# Autodesk Inventor assembly: ASSY,ROBOT,2026
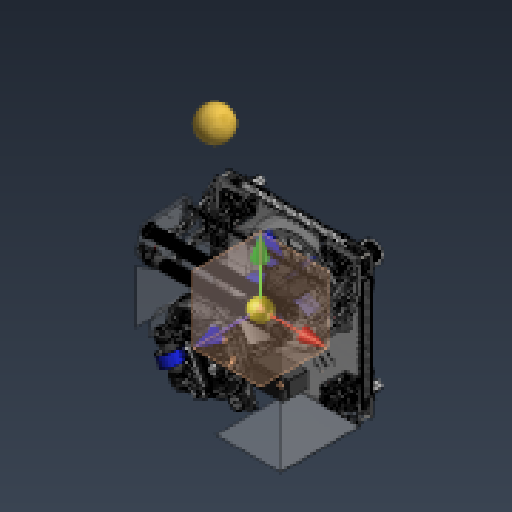
[picture p0: Inventor's stored thumbnail of the model, 512x512]
Saved by Autodesk Inventor 2026 (Build 300175050, 175E)
## iProperties
Created: 2026-01-24
Part Number: ASSY,ROBOT,2026
Document SubType Name: Assembly
Designer: Jthib
Mass: 50454.4 g
Surface Area: 114808 cm^2
Volume: 25614.5 cm^3
Density: 1.96976 g/cm^3
Author: Jthib
## Documents named in this file (11)
- C:\Users\Jthib\Documents\GitHub\2026-Robot-Mechanical\ASSY,ROBOT,2026.iam
- C:\Users\Jthib\Documents\GitHub\2026-Robot-Mechanical\Chassis\CHASSIS.iam
- C:\Users\Jthib\Documents\GitHub\2026-Robot-Mechanical\Spindexer\#Spindexer.iam
- C:\Users\Jthib\Documents\GitHub\2026-Robot-Mechanical\Shooter\Shooter - Front Motors\#SHOOTER.FRONT_MOTORS.iam
- C:\Users\Jthib\Documents\GitHub\2026-Robot-Mechanical\Shooter\Turret\#Turret.iam
- C:\Users\Jthib\Documents\GitHub\2026-Robot-Mechanical\Intake\ASSY,INTAKE.iam
- C:\Users\Jthib\Documents\GitHub\2026-Robot-Mechanical\#2_2026 Field CAD\GE-26900_ Fuel.ipt
- C:\Users\Jthib\Documents\GitHub\2026-Robot-Mechanical\Intake\PLATE,HOPPER,BACK.ipt
- C:\Users\Jthib\Documents\GitHub\2026-Robot-Mechanical\Intake\PLATE,HOPPER,FRONT.ipt
- C:\Users\Jthib\Documents\GitHub\2026-Robot-Mechanical\Intake\PLATE,HOPPER,BACK2.ipt
- C:\Users\Jthib\Documents\GitHub\2026-Robot-Mechanical\#1_CAD Library\Motors\MOTOR,REV,NEO,V1-1.ipt
## Components (11 placed, 10 different names)
1. CHASSIS:1 [sub-assembly] — Flush:1, Flush:2, Flush:3, Mate:9, Mate:10, Mate:11, Tangent:1, Mate:13, Mate:18, Mate:19, Mate:20, Mate:21, Flush:23, Mate:22, Flush:24, Mate:23, Mate:25, Flush:25
2. #Spindexer:1 [sub-assembly] — Mate:11, Mate:12, Tangent:1, Mate:13, Mate:15, Mate:16, Mate:17, Mate:18
3. #SHOOTER.FRONT_MOTORS:1 [sub-assembly] — Mate:9, Mate:10, Mate:12, Insert:1, Mate:14
4. #Turret:1 [sub-assembly] — Insert:1, Mate:14, Mate:15, Mate:16, Mate:17
5. ASSY,INTAKE:1 [sub-assembly] — Mate:19, Mate:20, Mate:21, Insert:2, Insert:3
6. GE-26900_ Fuel:1
7. PLATE,HOPPER,BACK:1 — Flush:23, Mate:22, Flush:24, Mate:24
8. PLATE,HOPPER,FRONT:1 — Mate:23, Mate:24
9. PLATE,HOPPER,BACK2:1 — Mate:25, Flush:25
10. MOTOR,REV,NEO,V1-1:1 — Insert:2
11. MOTOR,REV,NEO,V1-1:2 — Insert:3
## Relationships (27: Mate 17, Flush 6, Insert 3, Tangent 1)
- Flush:1 (-349.25 mm): CHASSIS:1
- Flush:2 (349.25 mm): CHASSIS:1
- Flush:3: CHASSIS:1
- Mate:9 (-190.5 mm): CHASSIS:1 ↔ #SHOOTER.FRONT_MOTORS:1
- Mate:10 (-190.5 mm): CHASSIS:1 ↔ #SHOOTER.FRONT_MOTORS:1
- Mate:11: CHASSIS:1 ↔ #Spindexer:1
- Mate:12 (79.375 mm): #Spindexer:1 ↔ #SHOOTER.FRONT_MOTORS:1
- Tangent:1: CHASSIS:1 ↔ #Spindexer:1
- Mate:13 (-304.8 mm): CHASSIS:1 ↔ #Spindexer:1
- Insert:1: #SHOOTER.FRONT_MOTORS:1 ↔ #Turret:1
- Mate:14: #SHOOTER.FRONT_MOTORS:1 ↔ #Turret:1
- Mate:15: #Spindexer:1 ↔ #Turret:1
- Mate:16: #Spindexer:1 ↔ #Turret:1
- Mate:17: #Spindexer:1 ↔ #Turret:1
- Mate:18: CHASSIS:1 ↔ #Spindexer:1
- Mate:19: CHASSIS:1 ↔ ASSY,INTAKE:1
- Mate:20: CHASSIS:1 ↔ ASSY,INTAKE:1
- Mate:21: CHASSIS:1 ↔ ASSY,INTAKE:1
- Flush:23: CHASSIS:1 ↔ PLATE,HOPPER,BACK:1
- Mate:22: CHASSIS:1 ↔ PLATE,HOPPER,BACK:1
- Flush:24: CHASSIS:1 ↔ PLATE,HOPPER,BACK:1
- Mate:23: CHASSIS:1 ↔ PLATE,HOPPER,FRONT:1
- Mate:24: PLATE,HOPPER,BACK:1 ↔ PLATE,HOPPER,FRONT:1
- Mate:25: CHASSIS:1 ↔ PLATE,HOPPER,BACK2:1
- Flush:25: CHASSIS:1 ↔ PLATE,HOPPER,BACK2:1
- Insert:2: ASSY,INTAKE:1 ↔ MOTOR,REV,NEO,V1-1:1
- Insert:3: ASSY,INTAKE:1 ↔ MOTOR,REV,NEO,V1-1:2
